# Autodesk Inventor assembly: RT_ARM_A_001
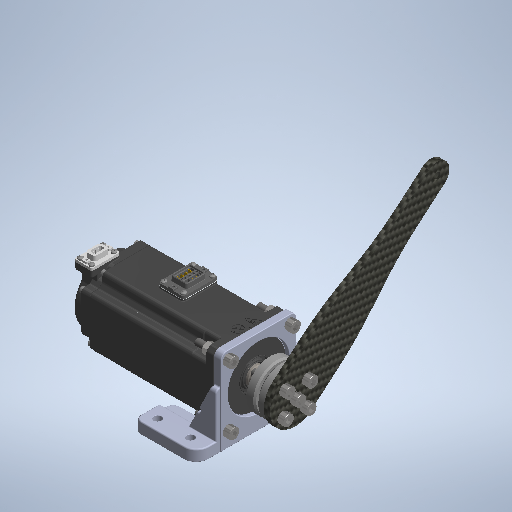
[picture p0: Inventor's stored thumbnail of the model, 512x512]
Saved by Autodesk Inventor 2025.4 (Build 294407000, 407)
## iProperties
Part Number: RT_ARM_A_001
Document SubType Name: Assembly
Designer: louis
Author: louis
## Documents named in this file (7)
- C:\Users\louis\OneDrive\Desktop\R_Trident\02_CAD\04_Subassemblies\RT_ARM_A_001.iam
- C:\Users\louis\OneDrive\Desktop\R_Trident\02_CAD\03_Parts_Custom\RT_ARM_MC_002.ipt
- C:\Users\louis\OneDrive\Desktop\R_Trident\02_CAD\01_Standard_Parts\A6M60-400H2B1-M17\A6M60-400H2B1-M17.iam
- C:\Users\louis\OneDrive\Desktop\R_Trident\02_CAD\01_Standard_Parts\ST-M4\ST-M4.ipt
- C:\Users\louis\OneDrive\Documents\Inventor\Content Center Files\R2025\en-US\ISO 4762(2)\ISO 4762 - M5 x 25ISO.ipt
- C:\Users\louis\OneDrive\Documents\Inventor\Content Center Files\R2025\en-US\ISO 4032(2)\ISO 4032 - M5 - ISO.ipt
- C:\Users\louis\OneDrive\Desktop\R_Trident\02_CAD\01_Standard_Parts\615 814 00\61581400.iam
## Components (17 placed, 6 different names)
1. 61581400:1 [sub-assembly] — Mate:20, Flush:2, Mate:21, Mate:22
2. ISO 4762 M5 x 25:5 — Insert:9
3. ISO 4762 M5 x 25:6 — Insert:10
4. ISO 4762 M5 x 25:8 — Insert:12
5. ISO 4762 M5 x 25:9 — Insert:13
6. ISO 4762 M5 x 25:10 — Insert:14
7. RT_ARM_MC_002:1 — Mate:21, Mate:22, Insert:9, Insert:10, Insert:12, Insert:13, Insert:14
8. A6M60-400H2B1-M17:1 [sub-assembly] — Mate:15, Mate:16, Mate:17, Insert:5, Insert:6, Insert:7, Insert:8, Flush:1, Mate:19, Mate:20, Flush:2
9. ST-M4:1 — Mate:15, Mate:16, Mate:17, Mate:18, Insert:1, Insert:2, Insert:3, Insert:4
10. ISO 4762 M5 x 25:1 — Insert:1
11. ISO 4762 M5 x 25:2 — Insert:2
12. ISO 4762 M5 x 25:3 — Insert:3
13. ISO 4762 M5 x 25:4 — Insert:4
14. ISO 4032 M5:1 — Insert:5
15. ISO 4032 M5:2 — Insert:6
16. ISO 4032 M5:3 — Insert:7
17. ISO 4032 M5:4 — Insert:8
## Relationships (23: Insert 13, Mate 8, Flush 2)
- Mate:15: A6M60-400H2B1-M17:1 ↔ ST-M4:1
- Mate:16: A6M60-400H2B1-M17:1 ↔ ST-M4:1
- Mate:17: A6M60-400H2B1-M17:1 ↔ ST-M4:1
- Mate:18: ST-M4:1
- Insert:1: ST-M4:1 ↔ ISO 4762 M5 x 25:1
- Insert:2: ST-M4:1 ↔ ISO 4762 M5 x 25:2
- Insert:3: ST-M4:1 ↔ ISO 4762 M5 x 25:3
- Insert:4: ST-M4:1 ↔ ISO 4762 M5 x 25:4
- Insert:5: A6M60-400H2B1-M17:1 ↔ ISO 4032 M5:1
- Insert:6: A6M60-400H2B1-M17:1 ↔ ISO 4032 M5:2
- Insert:7: A6M60-400H2B1-M17:1 ↔ ISO 4032 M5:3
- Insert:8: A6M60-400H2B1-M17:1 ↔ ISO 4032 M5:4
- Flush:1: A6M60-400H2B1-M17:1
- Mate:19: A6M60-400H2B1-M17:1
- Mate:20: 61581400:1 ↔ A6M60-400H2B1-M17:1
- Flush:2: 61581400:1 ↔ A6M60-400H2B1-M17:1
- Mate:21: 61581400:1 ↔ RT_ARM_MC_002:1
- Mate:22: 61581400:1 ↔ RT_ARM_MC_002:1
- Insert:9: ISO 4762 M5 x 25:5 ↔ RT_ARM_MC_002:1
- Insert:10: ISO 4762 M5 x 25:6 ↔ RT_ARM_MC_002:1
- Insert:12: ISO 4762 M5 x 25:8 ↔ RT_ARM_MC_002:1
- Insert:13: ISO 4762 M5 x 25:9 ↔ RT_ARM_MC_002:1
- Insert:14: ISO 4762 M5 x 25:10 ↔ RT_ARM_MC_002:1
